# Autodesk Inventor assembly: mg996r_motor_with_screws
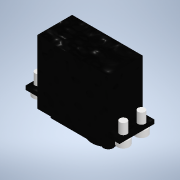
[picture p0: Inventor's stored thumbnail of the model, 180x180]
Saved by Autodesk Inventor 2021.4 (Build 254397000, 397)
## iProperties
Created: 2022-07-24
Part Number: mg996r_motor_with_screws
Document SubType Name: Assembly
Designer: isamu
Author: isamu
## Documents named in this file (3)
- D:\personal_projects\robot\inventor\2021_export_exp\mg996r_motor_with_screws.iam
- D:\personal_projects\robot\exports\servo motors\servo-motor-mg996r servo.ipt
- D:\personal_projects\robot\exports\screws\m4x8.ipt
## Components (5 placed, 2 different names)
1. servo-motor-mg996r servo:1 — Insert:1, Insert:2, Insert:3, Insert:4
2. m4x8:1 — Insert:2
3. m4x8:2 — Insert:1
4. m4x8:3 — Insert:3
5. m4x8:4 — Insert:4
## Relationships (4: Insert 4)
- Insert:1: servo-motor-mg996r servo:1 ↔ m4x8:2
- Insert:2: servo-motor-mg996r servo:1 ↔ m4x8:1
- Insert:3: servo-motor-mg996r servo:1 ↔ m4x8:3
- Insert:4: servo-motor-mg996r servo:1 ↔ m4x8:4
